# Autodesk Inventor assembly: Y_Mount_V2
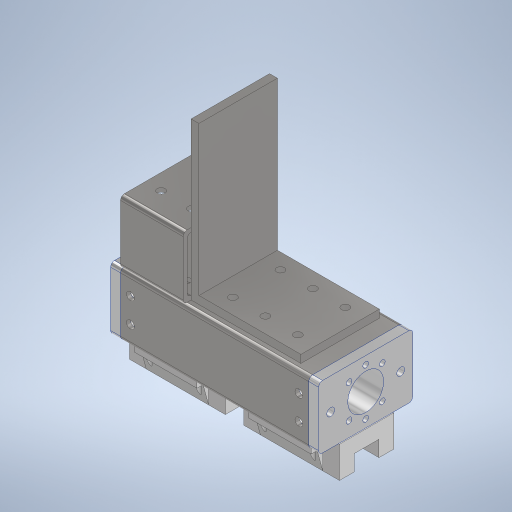
[picture p0: Inventor's stored thumbnail of the model, 512x512]
Saved by Autodesk Inventor 2023 (Build 270158000, 158)
## iProperties
Created: 2025-04-19
Part Number: Y_Mount_V2
Document SubType Name: Assembly
Designer: plebbb
Author: plebbb
## Documents named in this file (7)
- C:\Users\plebbb\Desktop\CNC_Project\Y_Mount_V2\Y_Mount_V2.iam
- C:\Users\plebbb\Desktop\CNC_Project\Y_Mount_V2\3x6_Bar.ipt
- C:\Users\plebbb\Desktop\CNC_Project\Y_Mount_V2\3x2_Bar.ipt
- C:\Users\plebbb\Desktop\CNC_Project\Y_Mount_V2\L_Channel.ipt
- C:\Users\plebbb\Desktop\CNC_Project\HGW20CC_Slider.ipt
- C:\Users\plebbb\Desktop\CNC_Project\Y_Mount_V2\BS_Face.ipt
- C:\Users\plebbb\Desktop\CNC_Project\SFU1605_Nut.ipt
## Components (8 placed, 6 different names)
1. 3x6_Bar:1 — Mate:1, Flush:1, Flush:2, Flush:3, Mate:2, Mate:4, Mate:5, Mate:6, Mate:7, Mate:8, Mate:9, Mate:10, Mate:11, Mate:12, Mate:16, Mate:17, Mate:18
2. 3x2_Bar:1 — Mate:1, Flush:1, Flush:2, Mate:3
3. L_Channel:1 — Flush:3, Mate:2, Mate:3
4. HGW20CC_Slider:1 — Mate:4, Mate:5, Mate:6
5. HGW20CC_Slider:2 — Mate:7, Mate:8, Mate:9
6. BS_Face:1 — Mate:10, Mate:11, Mate:12, Mate:13, Mate:14, Mate:15
7. SFU1605_Nut:1 — Mate:13, Mate:14, Mate:15
8. BS_Face:2 — Mate:16, Mate:17, Mate:18
## Relationships (21: Mate 18, Flush 3)
- Mate:1: 3x6_Bar:1 ↔ 3x2_Bar:1
- Flush:1: 3x6_Bar:1 ↔ 3x2_Bar:1
- Flush:2: 3x6_Bar:1 ↔ 3x2_Bar:1
- Flush:3 (6.35 mm): 3x6_Bar:1 ↔ L_Channel:1
- Mate:2: 3x6_Bar:1 ↔ L_Channel:1
- Mate:3: 3x2_Bar:1 ↔ L_Channel:1
- Mate:4: 3x6_Bar:1 ↔ HGW20CC_Slider:1
- Mate:5: 3x6_Bar:1 ↔ HGW20CC_Slider:1
- Mate:6: 3x6_Bar:1 ↔ HGW20CC_Slider:1
- Mate:7: 3x6_Bar:1 ↔ HGW20CC_Slider:2
- Mate:8: 3x6_Bar:1 ↔ HGW20CC_Slider:2
- Mate:9: 3x6_Bar:1 ↔ HGW20CC_Slider:2
- Mate:10: 3x6_Bar:1 ↔ BS_Face:1
- Mate:11: 3x6_Bar:1 ↔ BS_Face:1
- Mate:12: 3x6_Bar:1 ↔ BS_Face:1
- Mate:13: BS_Face:1 ↔ SFU1605_Nut:1
- Mate:14: BS_Face:1 ↔ SFU1605_Nut:1
- Mate:15: BS_Face:1 ↔ SFU1605_Nut:1
- Mate:16: 3x6_Bar:1 ↔ BS_Face:2
- Mate:17: 3x6_Bar:1 ↔ BS_Face:2
- Mate:18: 3x6_Bar:1 ↔ BS_Face:2
